# Autodesk Inventor assembly: Shoulder Joint Assembly
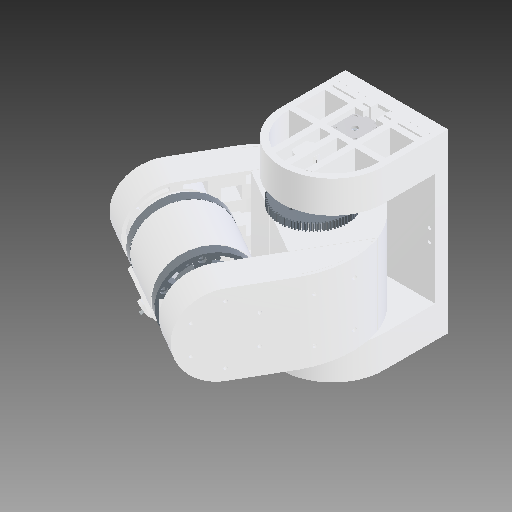
[picture p0: Inventor's stored thumbnail of the model, 512x512]
Saved by Autodesk Inventor 2017 SP1 (Build 210196100, 196)
## iProperties
Created: 2017-06-01
Part Number: Shoulder Joint Assembly
Document SubType Name: Assembly
Designer: Zach
Author: Zach
## Documents named in this file (17)
- C:\Users\Zach\Documents\GitHub\cr-laundry-robot\src\Body\Arm Assembly\Shoulder Joint Assembly\Shoulder Joint Assembly.iam
- C:\Users\Zach\Documents\GitHub\cr-laundry-robot\src\Body\Arm Assembly\Shoulder Joint Assembly\SJ002.ipt
- C:\Users\Zach\Documents\GitHub\cr-laundry-robot\src\Body\Arm Assembly\Shoulder Joint Assembly\SJ003.ipt
- C:\Users\Zach\Documents\GitHub\cr-laundry-robot\src\Body\Arm Assembly\Shoulder Joint Assembly\MC001.ipt
- C:\Users\Zach\Documents\GitHub\cr-laundry-robot\src\Body\Arm Assembly\Shoulder Joint Assembly\SJ001.ipt
- C:\Users\Zach\Documents\GitHub\cr-laundry-robot\src\Body\Arm Assembly\Shoulder Joint Assembly\MC002.ipt
- C:\Users\Zach\Documents\GitHub\cr-laundry-robot\lib\Stepper Motor - NEMA 17\NEMA17.ipt
- C:\Users\Zach\Documents\GitHub\cr-laundry-robot\src\Body\Arm Assembly\Shoulder Joint Assembly\SJ004.ipt
- C:\Users\Zach\Documents\GitHub\cr-laundry-robot\src\Body\Arm Assembly\Shoulder Joint Assembly\SJ005.ipt
- C:\Users\Zach\Documents\GitHub\cr-laundry-robot\src\Body\Arm Assembly\Shoulder Joint Assembly\SJ006.ipt
- C:\Users\Zach\Documents\GitHub\cr-laundry-robot\lib\U51105\U51105.ipt
- C:\Users\Zach\Documents\GitHub\cr-laundry-robot\lib\QS12MM250\QS12MM250.ipt
- C:\Users\Zach\Documents\GitHub\cr-laundry-robot\lib\6201RS\6201RS.ipt
- C:\Users\Zach\Documents\GitHub\cr-laundry-robot\src\Body\Arm Assembly\Shoulder Joint Assembly\SJ007.ipt
- C:\Users\Zach\Documents\GitHub\cr-laundry-robot\src\Body\Arm Assembly\Shoulder Joint Assembly\SJ008.ipt
- C:\Users\Zach\Documents\GitHub\cr-laundry-robot\src\Body\Arm Assembly\Shoulder Joint Assembly\Shoulder Joint Assembly\Design Accelerator\Spur Gears1.iam
- C:\Users\Zach\Documents\GitHub\cr-laundry-robot\src\Body\Arm Assembly\Shoulder Joint Assembly\SJ009.ipt
## Components (30 placed, 16 different names)
1. MC001:1 — Mate:5, Mate:6, Mate:7, Mate:27, Mate:32
2. MC001:2 — Mate:41, Mate:42
3. SJ002:1 — Mate:1, Mate:4, Mate:5, Mate:6, Mate:7, Mate:8, Mate:9
4. SJ002:2 — Mate:18, Mate:19, Mate:20
5. SJ003:1 — Mate:1, Mate:4, Mate:8, Mate:9, Mate:18, Mate:19, Mate:20, Mate:71, Mate:72, Mate:73
6. SJ001:1 — Mate:23, Mate:24, Mate:25, Mate:44, Mate:47, Mate:48, Mate:49
7. MC002:1 — Mate:23, Mate:24, Mate:25, Mate:27, Mate:28, Mate:29, Mate:30, Mate:31
8. NEMA17:1 — Mate:28, Mate:29, Mate:30, Mate:31, Mate:32
9. SJ001:2 — Mate:37, Mate:38, Mate:39, Mate:45, Mate:46
10. MC002:2 — Mate:33, Mate:35, Mate:37, Mate:38, Mate:39, Mate:40, Mate:41
11. NEMA17:2 — Mate:33, Mate:35, Mate:40, Mate:42
12. SJ004:1 — Mate:44, Mate:45, Mate:46, Mate:129, Mate:130, Mate:140, Mate:141
13. SJ004:2 — Mate:47, Mate:48, Mate:49, Mate:54, Mate:55, Mate:56, Mate:142, Mate:143
14. SJ005:1 — Mate:54, Mate:55, Mate:56, Mate:60, Mate:67, Mate:69, Mate:70, Mate:80
15. SJ005:2 — Mate:68, Mate:82, Mate:84, Mate:129, Mate:130, Mate:135, Mate:136
16. SJ006:2 — Mate:67, Mate:68, Mate:69, Mate:70, Mate:78, Mate:79, Mate:83
17. NEMA17:3 — Mate:71, Mate:72, Mate:73
18. U51105:1 — Mate:131, Mate:139
19. U51105:2 — Mate:78, Mate:79
20. QS12MM250:1 — Mate:80, Mate:105, Mate:117, Mate:119, Mate:120, Mate:132, Mate:134
21. 6201RS:1 — Mate:82, Mate:138
22. 6201RS:2 — Mate:83, Mate:84
23. SJ007:1 — Mate:121, Mate:122, Mate:123, Mate:133
24. SJ008:1 — Mate:119, Mate:125, Mate:126, Mate:127, Mate:132
25. SJ008:2 — Mate:97, Mate:98, Mate:99, Mate:105, Mate:112, Mate:117, Mate:120, Mate:121, Mate:122, Mate:123, Mate:124, Mate:131
26. NEMA17:4 — Mate:97, Mate:98, Mate:99, Mate:137
27. SJ007:2 — Mate:125, Mate:126, Mate:127, Mate:133
28. Spur Gears:1 [sub-assembly] — Mate:134, Mate:135, Mate:136, Mate:137, Mate:138, Mate:139
29. SJ009:1 — Mate:140, Mate:141
30. SJ009:2 — Mate:142, Mate:143
## Relationships (83: Mate 83)
- Mate:1: SJ002:1 ↔ SJ003:1
- Mate:4: SJ002:1 ↔ SJ003:1
- Mate:5: MC001:1 ↔ SJ002:1
- Mate:6: MC001:1 ↔ SJ002:1
- Mate:7: MC001:1 ↔ SJ002:1
- Mate:8: SJ002:1 ↔ SJ003:1
- Mate:9: SJ002:1 ↔ SJ003:1
- [Mate]: MC001:2 ↔ SJ002:2
- [Mate]: MC001:2 ↔ SJ002:2
- [Mate]: MC001:2 ↔ SJ002:2
- Mate:18: SJ002:2 ↔ SJ003:1
- Mate:19: SJ002:2 ↔ SJ003:1
- Mate:20: SJ002:2 ↔ SJ003:1
- Mate:23: SJ001:1 ↔ MC002:1
- Mate:24: SJ001:1 ↔ MC002:1
- Mate:25: SJ001:1 ↔ MC002:1
- Mate:27: MC001:1 ↔ MC002:1
- Mate:28: MC002:1 ↔ NEMA17:1
- Mate:29: MC002:1 ↔ NEMA17:1
- Mate:30: MC002:1 ↔ NEMA17:1
- Mate:31: MC002:1 ↔ NEMA17:1
- Mate:32: MC001:1 ↔ NEMA17:1
- Mate:33: MC002:2 ↔ NEMA17:2
- Mate:35: MC002:2 ↔ NEMA17:2
- Mate:37: SJ001:2 ↔ MC002:2
- Mate:38: SJ001:2 ↔ MC002:2
- Mate:39: SJ001:2 ↔ MC002:2
- Mate:40: MC002:2 ↔ NEMA17:2
- Mate:41: MC001:2 ↔ MC002:2
- Mate:42: MC001:2 ↔ NEMA17:2
- Mate:44: SJ001:1 ↔ SJ004:1
- Mate:45: SJ001:2 ↔ SJ004:1
- Mate:46: SJ001:2 ↔ SJ004:1
- Mate:47: SJ001:1 ↔ SJ004:2
- Mate:48: SJ001:1 ↔ SJ004:2
- Mate:49: SJ001:1 ↔ SJ004:2
- Mate:54: SJ004:2 ↔ SJ005:1
- Mate:55: SJ004:2 ↔ SJ005:1
- Mate:56: SJ004:2 ↔ SJ005:1
- Mate:60: SJ005:1
- Mate:67: SJ005:1 ↔ SJ006:2
- Mate:68: SJ005:2 ↔ SJ006:2
- Mate:69: SJ005:1 ↔ SJ006:2
- Mate:70: SJ005:1 ↔ SJ006:2
- Mate:71: SJ003:1 ↔ NEMA17:3
- Mate:72: SJ003:1 ↔ NEMA17:3
- Mate:73: SJ003:1 ↔ NEMA17:3
- Mate:78: SJ006:2 ↔ U51105:2
- Mate:79: SJ006:2 ↔ U51105:2
- Mate:80: SJ005:1 ↔ QS12MM250:1
- Mate:82: SJ005:2 ↔ 6201RS:1
- Mate:83: SJ006:2 ↔ 6201RS:2
- Mate:84: SJ005:2 ↔ 6201RS:2
- Mate:97: SJ008:2 ↔ NEMA17:4
- Mate:98: SJ008:2 ↔ NEMA17:4
- Mate:99: SJ008:2 ↔ NEMA17:4
- Mate:105: QS12MM250:1 ↔ SJ008:2
- Mate:112: SJ008:2
- Mate:117: QS12MM250:1 ↔ SJ008:2
- Mate:119: QS12MM250:1 ↔ SJ008:1
- Mate:120: QS12MM250:1 ↔ SJ008:2
- Mate:121: SJ007:1 ↔ SJ008:2
- Mate:122: SJ007:1 ↔ SJ008:2
- Mate:123: SJ007:1 ↔ SJ008:2
- Mate:124: SJ008:2
- Mate:125: SJ008:1 ↔ SJ007:2
- Mate:126: SJ008:1 ↔ SJ007:2
- Mate:127: SJ008:1 ↔ SJ007:2
- Mate:129: SJ004:1 ↔ SJ005:2
- Mate:130: SJ004:1 ↔ SJ005:2
- Mate:131: U51105:1 ↔ SJ008:2
- Mate:132: QS12MM250:1 ↔ SJ008:1
- Mate:133: SJ007:1 ↔ SJ007:2
- Mate:134: QS12MM250:1 ↔ Spur Gears:1
- Mate:135: SJ005:2 ↔ Spur Gears:1
- Mate:136: SJ005:2 ↔ Spur Gears:1
- Mate:137: NEMA17:4 ↔ Spur Gears:1
- Mate:138: 6201RS:1 ↔ Spur Gears:1
- Mate:139: U51105:1 ↔ Spur Gears:1
- Mate:140: SJ004:1 ↔ SJ009:1
- Mate:141: SJ004:1 ↔ SJ009:1
- Mate:142: SJ004:2 ↔ SJ009:2
- Mate:143: SJ004:2 ↔ SJ009:2
## Named parameters: d15_d4 = 0 mm, d16_d5 = 0 mm, d17_d7 = 0 mm
